# Autodesk Inventor assembly: Touch Segment
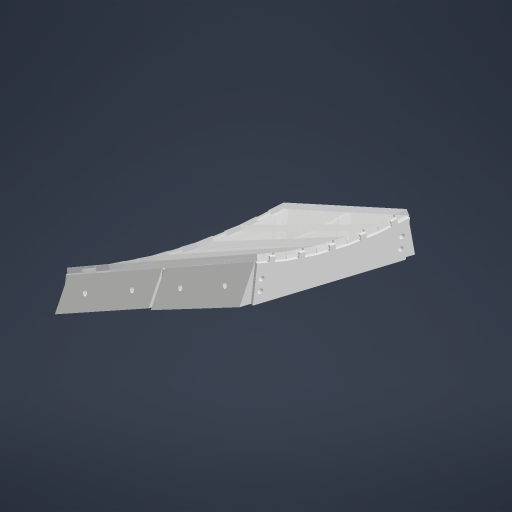
[picture p0: Inventor's stored thumbnail of the model, 512x512]
Saved by Autodesk Inventor 2023 (Build 270158000, 158)
## iProperties
Created: 2022-06-12
Part Number: Touch Segment
Document SubType Name: Assembly
Designer: FizzyApple12
Author: FizzyApple12
## Documents named in this file (9)
- C:\Users\FizzyApple12\Desktop\Wacca Controller V2\Touch Segment\Touch Segment.iam
- C:\Users\FizzyApple12\Desktop\Wacca Controller V2\Touch Segment\Touch Fifth.ipt
- C:\Users\FizzyApple12\Desktop\Wacca Controller V2\Touch Segment\Back Plate.ipt
- C:\Users\FizzyApple12\Desktop\Wacca Controller V2\Touch Segment\Front Plate.ipt
- C:\Users\FizzyApple12\Desktop\Wacca Controller V2\Touch Segment\Center Plate.ipt
- C:\Users\FizzyApple12\Desktop\Wacca Controller V2\Touch Segment\Upper Right Linkage.ipt
- C:\Users\FizzyApple12\Desktop\Wacca Controller V2\Touch Segment\Upper Left Linkage.ipt
- C:\Users\FizzyApple12\Desktop\Wacca Controller V2\Touch Segment\Inner Left Linkage.ipt
- C:\Users\FizzyApple12\Desktop\Wacca Controller V2\Touch Segment\Inner Right Linkage.ipt
## Components (12 placed, 8 different names)
1. Touch Fifth:1 — Mate:1, Mate:5, Flush:1, Mate:36, Mate:37, Mate:38, Flush:18, Mate:41, Flush:20, Flush:26
2. Touch Fifth:2 — Mate:1, Mate:2, Mate:5, Mate:6
3. Touch Fifth:3 — Mate:2, Mate:3, Mate:6, Mate:7, Mate:8, Mate:10, Flush:2, Mate:11, Flush:3, Mate:12
4. Touch Fifth:4 — Mate:3, Mate:4, Mate:7
5. Touch Fifth:5 — Mate:4, Mate:8, Flush:4, Mate:49
6. Back Plate:1 — Flush:1, Mate:10, Flush:16, Flush:17, Mate:39, Mate:40, Mate:45, Flush:21, Flush:22, Mate:48
7. Front Plate:1 — Flush:2, Mate:11
8. Center Plate:1 — Flush:3, Mate:12, Flush:4, Flush:19, Mate:46, Flush:23, Flush:24, Mate:47, Flush:25
9. Upper Left Linkage:1
10. Upper Right Linkage:1
11. Inner Left Linkage:1 — Flush:16, Mate:36, Mate:37, Mate:38, Flush:17, Flush:18, Mate:39, Mate:40, Mate:41, Flush:19, Flush:20, Mate:45, Mate:46, Flush:21, Flush:22, Flush:23, Flush:24, Flush:25, Flush:26
12. Inner Right Linkage:1 — Mate:47, Mate:48, Mate:49
## Relationships (63: Mate 37, Flush 26)
- Mate:1: Touch Fifth:1 ↔ Touch Fifth:2
- Mate:2: Touch Fifth:2 ↔ Touch Fifth:3
- Mate:3: Touch Fifth:3 ↔ Touch Fifth:4
- Mate:4: Touch Fifth:4 ↔ Touch Fifth:5
- Mate:5: Touch Fifth:1 ↔ Touch Fifth:2
- Mate:6: Touch Fifth:2 ↔ Touch Fifth:3
- Mate:7: Touch Fifth:3 ↔ Touch Fifth:4
- Mate:8: Touch Fifth:3 ↔ Touch Fifth:5
- Flush:1: Touch Fifth:1 ↔ Back Plate:1
- Mate:10: Touch Fifth:3 ↔ Back Plate:1
- Flush:2: Touch Fifth:3 ↔ Front Plate:1
- Mate:11: Touch Fifth:3 ↔ Front Plate:1
- Flush:3: Touch Fifth:3 ↔ Center Plate:1
- Mate:12: Touch Fifth:3 ↔ Center Plate:1
- Flush:4: Touch Fifth:5 ↔ Center Plate:1
- [Flush]: Center Plate:1 ↔ Upper Left Linkage:1
- [Mate]: Center Plate:1 ↔ Upper Left Linkage:1
- [Mate]: Center Plate:1 ↔ Upper Left Linkage:1
- [Mate]: Front Plate:1 ↔ Upper Left Linkage:1
- [Mate]: Front Plate:1 ↔ Upper Left Linkage:1
- [Mate]: Front Plate:1 ↔ Upper Left Linkage:1
- [Flush]: Touch Fifth:1 ↔ Upper Left Linkage:1
- [Flush]: Touch Fifth:1 ↔ Upper Left Linkage:1
- [Mate]: Touch Fifth:4 ↔ Upper Left Linkage:1
- [Mate]: Touch Fifth:4 ↔ Upper Left Linkage:1
- [Mate]: Touch Fifth:1 ↔ Upper Left Linkage:1
- [Mate]: Touch Fifth:1 ↔ Upper Left Linkage:1
- [Flush]: Front Plate:1 ↔ Upper Left Linkage:1
- [Flush]: Front Plate:1 ↔ Upper Left Linkage:1
- [Flush]: Front Plate:1 ↔ Upper Left Linkage:1
- [Flush]: Touch Fifth:1 ↔ Upper Left Linkage:1
- [Flush]: Center Plate:1 ↔ Upper Left Linkage:1
- [Flush]: Center Plate:1 ↔ Upper Left Linkage:1
- [Flush]: Center Plate:1 ↔ Upper Left Linkage:1
- [Flush]: Touch Fifth:1 ↔ Upper Left Linkage:1
- [Mate]: Touch Fifth:3 ↔ Upper Left Linkage:1
- [Mate]: Touch Fifth:3 ↔ Upper Left Linkage:1
- [Mate]: Touch Fifth:3 ↔ Upper Left Linkage:1
- [Mate]: Center Plate:1 ↔ Upper Right Linkage:1
- [Mate]: Front Plate:1 ↔ Upper Right Linkage:1
- [Mate]: Touch Fifth:5 ↔ Upper Right Linkage:1
- Flush:16: Back Plate:1 ↔ Inner Left Linkage:1
- Mate:36: Touch Fifth:1 ↔ Inner Left Linkage:1
- Mate:37: Touch Fifth:1 ↔ Inner Left Linkage:1
- Mate:38: Touch Fifth:1 ↔ Inner Left Linkage:1
- Flush:17: Back Plate:1 ↔ Inner Left Linkage:1
- Flush:18: Touch Fifth:1 ↔ Inner Left Linkage:1
- Mate:39: Back Plate:1 ↔ Inner Left Linkage:1
- Mate:40: Back Plate:1 ↔ Inner Left Linkage:1
- Mate:41: Touch Fifth:1 ↔ Inner Left Linkage:1
- Flush:19: Center Plate:1 ↔ Inner Left Linkage:1
- Flush:20: Touch Fifth:1 ↔ Inner Left Linkage:1
- Mate:45: Back Plate:1 ↔ Inner Left Linkage:1
- Mate:46: Center Plate:1 ↔ Inner Left Linkage:1
- Flush:21: Back Plate:1 ↔ Inner Left Linkage:1
- Flush:22: Back Plate:1 ↔ Inner Left Linkage:1
- Flush:23: Center Plate:1 ↔ Inner Left Linkage:1
- Flush:24: Center Plate:1 ↔ Inner Left Linkage:1
- Mate:47: Center Plate:1 ↔ Inner Right Linkage:1
- Mate:48: Back Plate:1 ↔ Inner Right Linkage:1
- Mate:49: Touch Fifth:5 ↔ Inner Right Linkage:1
- Flush:25: Center Plate:1 ↔ Inner Left Linkage:1
- Flush:26: Touch Fifth:1 ↔ Inner Left Linkage:1
